# Autodesk Inventor assembly: FGS
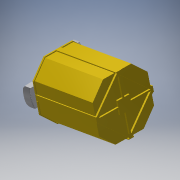
[picture p0: Inventor's stored thumbnail of the model, 180x180]
Saved by Autodesk Inventor 2018 (Build 220112000, 112)
## iProperties
Created: 2021-03-14
Part Number: FGS
Document SubType Name: Assembly
Designer: NITESH MAURYA
Author: NITESH MAURYA
## Documents named in this file (4)
- D:\Autodesk\Projects\C-C\ES101 GROUP-13 PROJECT\ES101 GROUP-13 PROJECT\FINAL MODEL\Resolved files\Assembly1.iam
- D:\Autodesk\Projects\C-C\ES101 GROUP-13 PROJECT\ES101 GROUP-13 PROJECT\INDIVIDUAL WORK\Nitesh\Resolved Parts\Derived FGS.ipt
- D:\Autodesk\Projects\C-C\ES101 GROUP-13 PROJECT\ES101 GROUP-13 PROJECT\INDIVIDUAL WORK\Nitesh\SupportingRod_CPY.ipt
- D:\Autodesk\Projects\C-C\ES101 GROUP-13 PROJECT\ES101 GROUP-13 PROJECT\INDIVIDUAL WORK\Tejas\Part1 - Instrument modules.ipt
## Components (7 placed, 3 different names)
1. Derived FGS:1 — Mate:12, Mate:16, Mate:21
2. Derived FGS:2 — Mate:16, Mate:17, Mate:20
3. Derived FGS:3 — Mate:18, Mate:19, Mate:20, Mate:21
4. SupportingRod_CPY:2 — Mate:9, Mate:13, Mate:18
5. SupportingRod_CPY:3 — Mate:10, Mate:12, Mate:15
6. Part1 - Instrument modules:1 — Mate:9, Mate:10, Mate:11, Mate:13, Mate:14, Mate:15, Mate:19
7. SupportingRod_CPY:4 — Mate:11, Mate:14, Mate:17
## Relationships (13: Mate 13)
- Mate:9 (-12.7 mm): SupportingRod_CPY:2 ↔ Part1 - Instrument modules:1
- Mate:10 (-12.7 mm): SupportingRod_CPY:3 ↔ Part1 - Instrument modules:1
- Mate:11 (-12.7 mm): Part1 - Instrument modules:1 ↔ SupportingRod_CPY:4
- Mate:12: Derived FGS:1 ↔ SupportingRod_CPY:3
- Mate:13 (50.8 mm): SupportingRod_CPY:2 ↔ Part1 - Instrument modules:1
- Mate:14 (50.8 mm): Part1 - Instrument modules:1 ↔ SupportingRod_CPY:4
- Mate:15 (50.8 mm): SupportingRod_CPY:3 ↔ Part1 - Instrument modules:1
- Mate:16 (20.32 mm): Derived FGS:1 ↔ Derived FGS:2
- Mate:17: Derived FGS:2 ↔ SupportingRod_CPY:4
- Mate:18: Derived FGS:3 ↔ SupportingRod_CPY:2
- Mate:19: Derived FGS:3 ↔ Part1 - Instrument modules:1
- Mate:20 (20.32 mm): Derived FGS:2 ↔ Derived FGS:3
- Mate:21 (20.32 mm): Derived FGS:1 ↔ Derived FGS:3
